# Autodesk Inventor assembly: onering_tire_set_2
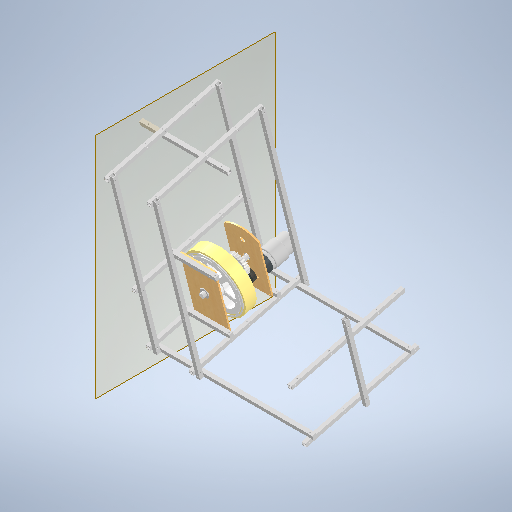
[picture p0: Inventor's stored thumbnail of the model, 512x512]
Saved by Autodesk Inventor 2025.1 (Build 291241000, 241)
## iProperties
Created: 2024-10-03
Part Number: onering_tire_set_2
Document SubType Name: Assembly
Designer: yuki0520
Author: yuki0520
## Documents named in this file (17)
- C:\Users\yuki0520\OneDrive\ドキュメント\Inventor\2025_nhk\tanaka\nageru\onering\onering_tire_set_2.iam
- C:\Users\yuki0520\OneDrive\ドキュメント\Inventor\2025_nhk\tanaka\nageru\pakuriz\tire.iam
- C:\Users\yuki0520\OneDrive\ドキュメント\Inventor\2025_nhk\tanaka\nageru\pakuriz\TH22_Bar_roller_sn.ipt
- C:\Users\yuki0520\OneDrive\ドキュメント\Inventor\2025_nhk\tanaka\inventorパーツリスト\モーター\775\RS-775GM.ipt
- C:\Users\yuki0520\OneDrive\ドキュメント\Inventor\2025_nhk\tanaka\inventorパーツリスト\モーター\775\RS-775GM_004GH_sn.ipt
- C:\Users\yuki0520\OneDrive\ドキュメント\Inventor\2025_nhk\tanaka\nageru\pakuriz\gear_kiseihin.iam
- C:\Users\yuki0520\OneDrive\ドキュメント\Inventor\2025_nhk\tanaka\nageru\pakuriz\bear_12_18.ipt
- C:\Users\yuki0520\OneDrive\ドキュメント\Inventor\2025_nhk\tanaka\nageru\onering\onering_plate_test.ipt
- C:\Users\yuki0520\OneDrive\ドキュメント\Inventor\2025_nhk\tanaka\nageru\onering\kaku_1010_425_onetire.ipt
- C:\Users\yuki0520\OneDrive\ドキュメント\Inventor\2025_nhk\tanaka\nageru\onering\onering_plate_test_nomotor.ipt
- C:\Users\yuki0520\OneDrive\ドキュメント\Inventor\2025_nhk\tanaka\nageru\pakuriz\TH22_Setcolor_12_sn.ipt
- C:\Users\yuki0520\OneDrive\ドキュメント\Inventor\2025_nhk\tanaka\nageru\onering\jik_motor_12_50.ipt
- C:\Users\yuki0520\OneDrive\ドキュメント\Inventor\2025_nhk\tanaka\nageru\onering\kaku_1010_145.ipt
- C:\Users\yuki0520\OneDrive\ドキュメント\Inventor\2025_nhk\tanaka\nageru\onering\kaku_1010_206_sororail.ipt
- C:\Users\yuki0520\OneDrive\ドキュメント\Inventor\2025_nhk\tanaka\nageru\onering\kaku_1010_onetire_plate.ipt
- C:\Users\yuki0520\OneDrive\ドキュメント\Inventor\2025_nhk\tanaka\nageru\onering\kaku_1010_206_sororail_2.ipt
- C:\Users\yuki0520\OneDrive\ドキュメント\Inventor\2025_nhk\tanaka\nageru\onering\kaku_1010_top_2.ipt
## Components (29 placed, 16 different names)
1. tire:1 [sub-assembly] — メイト:1, メイト:3, メイト:29
2. TH22_Bar_roller_sn:1 — メイト:1, メイト:3, メイト:11, メイト:15, メイト:16, メイト:17, メイト:20, メイト:21
3. RS-775GM:1 — メイト:4, 正接:1
4. RS-775GM_004GH_sn:1 — メイト:4, 正接:1, 挿入:1, メイト:25, メイト:26
5. gear_kiseihin:1 [sub-assembly] — メイト:11, メイト:20, メイト:28, メイト:31
6. bear_12_18:1 — メイト:15, メイト:22
7. bear_12_18:2 — メイト:16, メイト:19
8. onering_plate_test:1 — メイト:17, 挿入:1, メイト:19, メイト:27, メイト:30, 挿入:52, 挿入:53
9. onering_plate_test_nomotor:1 — メイト:21, メイト:22, メイト:29, 挿入:32, 挿入:33, 挿入:50, 挿入:51
10. TH22_Setcolor_12_sn:1 — メイト:27, メイト:32
11. jik_motor_12_50:1 — メイト:25, メイト:26, メイト:28, メイト:30, メイト:31, メイト:32
12. kaku_1010_145:1 — 挿入:46, 挿入:47, 挿入:58
13. kaku_1010_145:2 — 挿入:28, 挿入:48, 挿入:49
14. kaku_1010_206_sororail:1 — 挿入:28, 挿入:58
15. kaku_1010_onetire_plate:1 — 挿入:50, 挿入:51, 挿入:54, 挿入:64
16. kaku_1010_onetire_plate:3 — 挿入:32, 挿入:33, 挿入:59
17. kaku_1010_onetire_plate:4 — 挿入:52, 挿入:53, 挿入:55, 挿入:63
18. kaku_1010_145:3 — 挿入:42, 挿入:43, 挿入:63, 挿入:64, 挿入:85, 挿入:92, メイト:33
19. kaku_1010_145:4 — 挿入:44, 挿入:45, 挿入:54, 挿入:55, 挿入:87
20. kaku_1010_425_onetire:1 — 挿入:45, 挿入:49
21. kaku_1010_425_onetire:2 — 挿入:43, 挿入:46, 挿入:61, 挿入:86
22. kaku_1010_425_onetire:3 — 挿入:44, 挿入:48
23. kaku_1010_425_onetire:4 — 挿入:42, 挿入:47, 挿入:62, 挿入:93
24. kaku_1010_145:5 — 挿入:59, 挿入:61, 挿入:62
25. kaku_1010_145:6 — 挿入:83, 挿入:94, 挿入:95
26. kaku_1010_145:7 — 挿入:84
27. kaku_1010_206_sororail_2:1 — 挿入:83, 挿入:84
28. kaku_1010_top_2:1 — 挿入:85, 挿入:86, 挿入:87, 挿入:95
29. kaku_1010_top_2:4 — 挿入:92, 挿入:93, 挿入:94
## Relationships (54: Insert 33, Mate 20, Tangent 1)
- メイト:1 [Mate]: tire:1 ↔ TH22_Bar_roller_sn:1
- メイト:3 [Mate]: tire:1 ↔ TH22_Bar_roller_sn:1
- メイト:4 [Mate]: RS-775GM:1 ↔ RS-775GM_004GH_sn:1
- 正接:1 [Tangent]: RS-775GM:1 ↔ RS-775GM_004GH_sn:1
- メイト:11 [Mate]: TH22_Bar_roller_sn:1 ↔ gear_kiseihin:1
- メイト:15 [Mate]: TH22_Bar_roller_sn:1 ↔ bear_12_18:1
- メイト:16 [Mate]: TH22_Bar_roller_sn:1 ↔ bear_12_18:2
- メイト:17 [Mate]: TH22_Bar_roller_sn:1 ↔ onering_plate_test:1
- 挿入:1 [Insert]: RS-775GM_004GH_sn:1 ↔ onering_plate_test:1
- メイト:19 [Mate]: bear_12_18:2 ↔ onering_plate_test:1
- メイト:20 [Mate]: TH22_Bar_roller_sn:1 ↔ gear_kiseihin:1
- メイト:21 [Mate]: TH22_Bar_roller_sn:1 ↔ onering_plate_test_nomotor:1
- メイト:22 [Mate]: bear_12_18:1 ↔ onering_plate_test_nomotor:1
- メイト:25 [Mate]: RS-775GM_004GH_sn:1 ↔ jik_motor_12_50:1
- メイト:26 [Mate]: RS-775GM_004GH_sn:1 ↔ jik_motor_12_50:1
- メイト:27 [Mate]: onering_plate_test:1 ↔ TH22_Setcolor_12_sn:1
- メイト:28 [Mate]: gear_kiseihin:1 ↔ jik_motor_12_50:1
- メイト:29 [Mate]: tire:1 ↔ onering_plate_test_nomotor:1
- メイト:30 [Mate]: onering_plate_test:1 ↔ jik_motor_12_50:1
- メイト:31 [Mate]: gear_kiseihin:1 ↔ jik_motor_12_50:1
- メイト:32 [Mate]: TH22_Setcolor_12_sn:1 ↔ jik_motor_12_50:1
- 挿入:28 [Insert]: kaku_1010_145:2 ↔ kaku_1010_206_sororail:1
- 挿入:32 [Insert]: onering_plate_test_nomotor:1 ↔ kaku_1010_onetire_plate:3
- 挿入:33 [Insert]: onering_plate_test_nomotor:1 ↔ kaku_1010_onetire_plate:3
- 挿入:42 [Insert]: kaku_1010_145:3 ↔ kaku_1010_425_onetire:4
- 挿入:43 [Insert]: kaku_1010_145:3 ↔ kaku_1010_425_onetire:2
- 挿入:44 [Insert]: kaku_1010_145:4 ↔ kaku_1010_425_onetire:3
- 挿入:45 [Insert]: kaku_1010_145:4 ↔ kaku_1010_425_onetire:1
- 挿入:46 [Insert]: kaku_1010_145:1 ↔ kaku_1010_425_onetire:2
- 挿入:47 [Insert]: kaku_1010_145:1 ↔ kaku_1010_425_onetire:4
- 挿入:48 [Insert]: kaku_1010_145:2 ↔ kaku_1010_425_onetire:3
- 挿入:49 [Insert]: kaku_1010_145:2 ↔ kaku_1010_425_onetire:1
- 挿入:50 [Insert]: onering_plate_test_nomotor:1 ↔ kaku_1010_onetire_plate:1
- 挿入:51 [Insert]: onering_plate_test_nomotor:1 ↔ kaku_1010_onetire_plate:1
- 挿入:52 [Insert]: onering_plate_test:1 ↔ kaku_1010_onetire_plate:4
- 挿入:53 [Insert]: onering_plate_test:1 ↔ kaku_1010_onetire_plate:4
- 挿入:54 [Insert]: kaku_1010_onetire_plate:1 ↔ kaku_1010_145:4
- 挿入:55 [Insert]: kaku_1010_onetire_plate:4 ↔ kaku_1010_145:4
- 挿入:58 [Insert]: kaku_1010_145:1 ↔ kaku_1010_206_sororail:1
- 挿入:59 [Insert]: kaku_1010_onetire_plate:3 ↔ kaku_1010_145:5
- 挿入:61 [Insert]: kaku_1010_425_onetire:2 ↔ kaku_1010_145:5
- 挿入:62 [Insert]: kaku_1010_425_onetire:4 ↔ kaku_1010_145:5
- 挿入:63 [Insert]: kaku_1010_onetire_plate:4 ↔ kaku_1010_145:3
- 挿入:64 [Insert]: kaku_1010_onetire_plate:1 ↔ kaku_1010_145:3
- 挿入:83 [Insert]: kaku_1010_145:6 ↔ kaku_1010_206_sororail_2:1
- 挿入:84 [Insert]: kaku_1010_145:7 ↔ kaku_1010_206_sororail_2:1
- 挿入:85 [Insert]: kaku_1010_145:3 ↔ kaku_1010_top_2:1
- 挿入:86 [Insert]: kaku_1010_425_onetire:2 ↔ kaku_1010_top_2:1
- 挿入:87 [Insert]: kaku_1010_145:4 ↔ kaku_1010_top_2:1
- 挿入:92 [Insert]: kaku_1010_145:3 ↔ kaku_1010_top_2:4
- 挿入:93 [Insert]: kaku_1010_425_onetire:4 ↔ kaku_1010_top_2:4
- 挿入:94 [Insert]: kaku_1010_145:6 ↔ kaku_1010_top_2:4
- 挿入:95 [Insert]: kaku_1010_145:6 ↔ kaku_1010_top_2:1
- メイト:33 [Mate]: kaku_1010_145:3
